# Autodesk Inventor assembly: mg996r_left_top_rot_frame
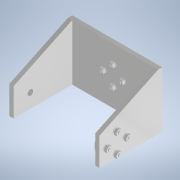
[picture p0: Inventor's stored thumbnail of the model, 180x180]
Saved by Autodesk Inventor 2021.4 (Build 254397000, 397)
## iProperties
Created: 2022-08-03
Part Number: mg996r_left_top_rot_frame
Document SubType Name: Assembly
Designer: isamu
Author: isamu
## Documents named in this file (6)
- D:\personal_projects\robot\inventor\2021_matlab_compat _v2\servo_rot_frame\mg996r_left_top_rot_frame.iam
- D:\personal_projects\robot\exports\frames\servo frame mg996 centered.ipt
- D:\personal_projects\robot\inventor\2021_matlab_compat _v2\servo_frames\servo_handle.iam
- D:\personal_projects\robot\exports\screws\m2 washer.ipt
- D:\personal_projects\robot\exports\screws\m2 nuts.ipt
- D:\personal_projects\robot\exports\screws\m4 nuts.ipt
## Components (20 placed, 5 different names)
1. servo frame mg996 centered:1 — Mate:1, Mate:2, Mate:3, Mate:4, Mate:5, Mate:6, Insert:1, Insert:2, Insert:3, Insert:4, Insert:9, Insert:10, Insert:11, Insert:12, Insert:13
2. servo_handle:1 [sub-assembly] — Mate:1, Mate:2, Mate:3
3. servo_handle:2 [sub-assembly] — Mate:4, Mate:5, Mate:6
4. m2 washer:1 — Insert:2, Insert:6
5. m2 washer:2 — Insert:1, Insert:5
6. m2 washer:3 — Insert:10, Insert:15
7. m2 washer:4 — Insert:12, Insert:16
8. m2 washer:5 — Insert:4, Insert:8
9. m2 washer:6 — Insert:3, Insert:7
10. m2 washer:7 — Insert:11, Insert:14
11. m2 washer:8 — Insert:13, Insert:17
12. m2 nuts:1 — Insert:15
13. m2 nuts:2 — Insert:8
14. m2 nuts:3 — Insert:6
15. m2 nuts:4 — Insert:5
16. m2 nuts:5 — Insert:7
17. m2 nuts:6 — Insert:14
18. m2 nuts:7 — Insert:16
19. m2 nuts:8 — Insert:17
20. m4 nuts:1 — Insert:9
## Relationships (23: Insert 17, Mate 6)
- Mate:1: servo frame mg996 centered:1 ↔ servo_handle:1
- Mate:2: servo frame mg996 centered:1 ↔ servo_handle:1
- Mate:3: servo frame mg996 centered:1 ↔ servo_handle:1
- Mate:4: servo frame mg996 centered:1 ↔ servo_handle:2
- Mate:5: servo frame mg996 centered:1 ↔ servo_handle:2
- Mate:6: servo frame mg996 centered:1 ↔ servo_handle:2
- Insert:1: servo frame mg996 centered:1 ↔ m2 washer:2
- Insert:2: servo frame mg996 centered:1 ↔ m2 washer:1
- Insert:3: servo frame mg996 centered:1 ↔ m2 washer:6
- Insert:4: servo frame mg996 centered:1 ↔ m2 washer:5
- Insert:5: m2 washer:2 ↔ m2 nuts:4
- Insert:6: m2 washer:1 ↔ m2 nuts:3
- Insert:7: m2 washer:6 ↔ m2 nuts:5
- Insert:8: m2 washer:5 ↔ m2 nuts:2
- Insert:9: servo frame mg996 centered:1 ↔ m4 nuts:1
- Insert:10: servo frame mg996 centered:1 ↔ m2 washer:3
- Insert:11: servo frame mg996 centered:1 ↔ m2 washer:7
- Insert:12: servo frame mg996 centered:1 ↔ m2 washer:4
- Insert:13: servo frame mg996 centered:1 ↔ m2 washer:8
- Insert:14: m2 washer:7 ↔ m2 nuts:6
- Insert:15: m2 washer:3 ↔ m2 nuts:1
- Insert:16: m2 washer:4 ↔ m2 nuts:7
- Insert:17: m2 washer:8 ↔ m2 nuts:8
